# Autodesk Inventor assembly: swerve but cooler full assembly
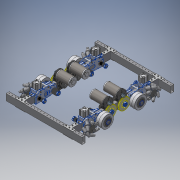
[picture p0: Inventor's stored thumbnail of the model, 180x180]
Saved by Autodesk Inventor 2018 (Build 220112000, 112)
## iProperties
Created: 2020-05-06
Part Number: swerve but cooler full assembly
Document SubType Name: Assembly
Designer: maste
Author: maste
## Documents named in this file (3)
- C:\Users\maste\OneDrive\Documents\GitHub\2020CAD\Offseason Stuff\swerve but cooler\Part Files\swerve but cooler full assembly.iam
- C:\Users\maste\OneDrive\Documents\GitHub\2020CAD\Offseason Stuff\swerve but cooler\Part Files\Driveline (belt edition).iam
- C:\Users\maste\OneDrive\Documents\GitHub\2020CAD\Offseason Stuff\swerve but cooler\Part Files\Front and Back Bar.ipt
## Components (4 placed, 2 different names)
1. Driveline (belt edition):1 [sub-assembly] — Mate:1, Flush:1, Mate:5, Flush:4
2. Driveline (belt edition):2 [sub-assembly] — Mate:2, Flush:3, Mate:4, Mate:6
3. Front and Back Bar:1 — Mate:1, Flush:1, Mate:2, Flush:3, Mate:6
4. Front and Back Bar:2 — Mate:4, Mate:5, Flush:4
## Relationships (8: Mate 5, Flush 3)
- Mate:1: Driveline (belt edition):1 ↔ Front and Back Bar:1
- Flush:1: Driveline (belt edition):1 ↔ Front and Back Bar:1
- Mate:2: Driveline (belt edition):2 ↔ Front and Back Bar:1
- Flush:3: Driveline (belt edition):2 ↔ Front and Back Bar:1
- Mate:4: Driveline (belt edition):2 ↔ Front and Back Bar:2
- Mate:5: Driveline (belt edition):1 ↔ Front and Back Bar:2
- Flush:4: Driveline (belt edition):1 ↔ Front and Back Bar:2
- Mate:6: Driveline (belt edition):2 ↔ Front and Back Bar:1
